# Autodesk Inventor assembly: Arm - Standalone
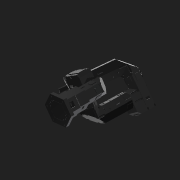
[picture p0: Inventor's stored thumbnail of the model, 180x180]
Saved by Autodesk Inventor 2017 (Build 210142000, 142)
## iProperties
Created: 2019-07-18
Part Number: Arm - Standalone
Document SubType Name: Assembly
Designer: Dell
Author: Dell
## Documents named in this file (8)
- C:\Users\Dell\Documents\GitHub\tr2\Arm - Standalone\Arm - Standalone.iam
- C:\Users\Dell\Documents\GitHub\tr2\Arm\TARM09b.ipt
- C:\Users\Dell\Documents\GitHub\tr2\Arm\TARM02b.ipt
- C:\Users\Dell\Documents\GitHub\tr2\Arm\TARM14.ipt
- C:\Users\Dell\Documents\GitHub\tr2\Actuator 1.3\Actuator 1.3.iam
- C:\Users\Dell\Documents\GitHub\tr2\Gripper 1.1\Gripper 1.1.iam
- C:\Users\Dell\Documents\GitHub\tr2\Arm\TARM15.ipt
- C:\Users\Dell\Documents\GitHub\tr2\Arm\TARM16.ipt
## Components (13 placed, 7 different names)
1. TARM09b:1
2. TARM09b:2
3. TARM02b:1
4. TARM14:1
5. TARM14:2
6. Actuator 1.3:1 [sub-assembly] — Mate:26, Mate:27, Mate:28, Mate:29
7. Actuator 1.3:2 [sub-assembly]
8. Actuator 1.3:3 [sub-assembly]
9. Actuator 1.3:4 [sub-assembly]
10. Actuator 1.3:5 [sub-assembly]
11. Gripper 1.1:1 [sub-assembly]
12. TARM15:1 — Mate:26, Mate:27, Mate:28, Mate:29, Mate:30, Mate:31, Mate:32
13. TARM16:1 — Mate:30, Mate:31, Mate:32
## Relationships (32: Mate 32)
- [Mate]: TARM09b:1 ↔ TARM02b:1
- [Mate]: TARM09b:1 ↔ TARM02b:1
- [Mate]: TARM09b:1 ↔ TARM02b:1
- [Mate]: TARM02b:1 ↔ Actuator 1.3:1
- [Mate]: TARM02b:1 ↔ Actuator 1.3:1
- [Mate]: TARM09b:1 ↔ Actuator 1.3:2
- [Mate]: TARM09b:1 ↔ Actuator 1.3:2
- [Mate]: TARM09b:1 ↔ Actuator 1.3:2
- [Mate]: TARM14:1 ↔ Actuator 1.3:2
- [Mate]: TARM14:1 ↔ Actuator 1.3:2
- [Mate]: TARM14:1 ↔ Actuator 1.3:3
- [Mate]: TARM14:1 ↔ Actuator 1.3:3
- [Mate]: TARM14:1 ↔ Actuator 1.3:3
- [Mate]: TARM09b:2 ↔ Actuator 1.3:3
- [Mate]: TARM09b:2 ↔ Actuator 1.3:3
- [Mate]: TARM09b:2 ↔ Actuator 1.3:4
- [Mate]: TARM09b:2 ↔ Actuator 1.3:4
- [Mate]: TARM09b:2 ↔ Actuator 1.3:4
- [Mate]: TARM14:2 ↔ Actuator 1.3:4
- [Mate]: TARM14:2 ↔ Actuator 1.3:4
- [Mate]: TARM14:2 ↔ Actuator 1.3:5
- [Mate]: TARM14:2 ↔ Actuator 1.3:5
- [Mate]: TARM14:2 ↔ Actuator 1.3:5
- [Mate]: Actuator 1.3:5 ↔ Gripper 1.1:1
- [Mate]: Actuator 1.3:5 ↔ Gripper 1.1:1
- Mate:26: Actuator 1.3:1 ↔ TARM15:1
- Mate:27: Actuator 1.3:1 ↔ TARM15:1
- Mate:28: Actuator 1.3:1 ↔ TARM15:1
- Mate:29: Actuator 1.3:1 ↔ TARM15:1
- Mate:30: TARM15:1 ↔ TARM16:1
- Mate:31: TARM15:1 ↔ TARM16:1
- Mate:32: TARM15:1 ↔ TARM16:1
